# Autodesk Inventor assembly: 1 by 4
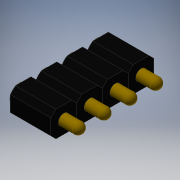
[picture p0: Inventor's stored thumbnail of the model, 180x180]
Saved by Autodesk Inventor 2016 (Build 200138000, 138)
## iProperties
Created: 2016-05-20
Part Number: 1 by 4
Document SubType Name: Assembly
Designer: Jonathan
Author: Jonathan
## Documents named in this file (3)
- C:\Users\sawaiz\oneDrive\projects\splitFlapDisplay\electronics\cad\component\Preci-Dip 811\1 by 4.iam
- C:\Users\sawaiz\oneDrive\projects\splitFlapDisplay\electronics\cad\component\Preci-Dip 811\body.ipt
- C:\Users\sawaiz\oneDrive\projects\splitFlapDisplay\electronics\cad\component\Preci-Dip 811\pin.ipt
## Components (8 placed, 2 different names)
1. body:1 — Mate:1, Mate:2, Flush:1
2. pin:1 — Mate:1, Mate:2, Flush:1
3. body:2
4. pin:2
5. body:3
6. pin:3
7. body:4
8. pin:4
## Component patterns: (4 elements, first: body:1 + pin:1)
## Relationships (3: Mate 2, Flush 1)
- Mate:1: body:1 ↔ pin:1
- Mate:2: body:1 ↔ pin:1
- Flush:1 (3.75 mm): body:1 ↔ pin:1
